# Autodesk Inventor assembly: mesa_0001_00001
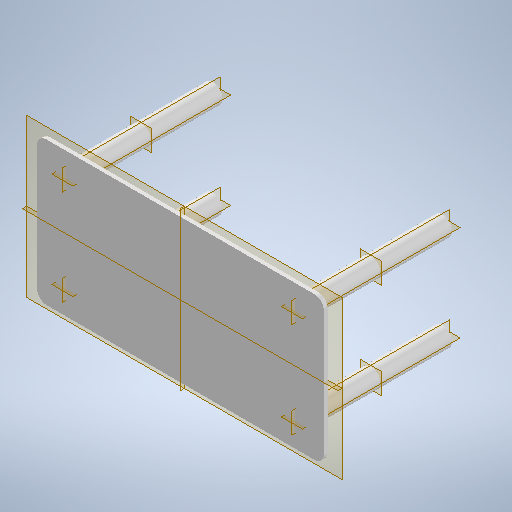
[picture p0: Inventor's stored thumbnail of the model, 512x512]
Saved by Autodesk Inventor 2025.2 (Build 292293000, 293)
## iProperties
Created: 2025-03-28
Part Number: mesa_0001_00001
Document SubType Name: Assembly
Designer: kenne
Author: kenne
## Documents named in this file (3)
- C:\Users\kenne\OneDrive\Ambiente de Trabalho\Robotica & Automação\Sistemas de Microcontroladores\Learning\Inventor\Exercices\Mesa\mesa_0001_00001.iam
- C:\Users\kenne\OneDrive\Ambiente de Trabalho\Robotica & Automação\Sistemas de Microcontroladores\Learning\Inventor\Exercices\Mesa\mesa_0001_00001.ipt
- C:\Users\kenne\OneDrive\Ambiente de Trabalho\Robotica & Automação\Sistemas de Microcontroladores\Learning\Inventor\Exercices\Mesa\pernas_0001_00001.ipt
## Components (5 placed, 2 different names)
1. mesa_0001_00001:1 — Flush:1, Flush:2, Flush:3, Mate:1, Flush:4, Flush:5
2. pernas_0001_00001:1 — Flush:7, Flush:9, Flush:10, Flush:11, Symmetry:1, Flush:14, Flush:15, Symmetry:2, Flush:16, Flush:17, Symmetry:3
3. pernas_0001_00001:2 — Flush:8, Flush:10, Flush:13, Flush:16, Symmetry:3
4. pernas_0001_00001:3 — Mate:1, Flush:4, Flush:5, Flush:6, Flush:7, Flush:8, Flush:12, Flush:13, Symmetry:1
5. pernas_0001_00001:4 — Flush:6, Flush:9, Flush:11, Flush:12, Flush:14, Flush:15, Symmetry:2, Flush:17
## Relationships (21: Flush 17, Symmetry 3, Mate 1)
- Flush:1: mesa_0001_00001:1
- Flush:2: mesa_0001_00001:1
- Flush:3: mesa_0001_00001:1
- Mate:1: mesa_0001_00001:1 ↔ pernas_0001_00001:3
- Flush:4 (600 mm): mesa_0001_00001:1 ↔ pernas_0001_00001:3
- Flush:5 (250 mm): mesa_0001_00001:1 ↔ pernas_0001_00001:3
- Flush:6: pernas_0001_00001:3 ↔ pernas_0001_00001:4
- Flush:7: pernas_0001_00001:1 ↔ pernas_0001_00001:3
- Flush:8: pernas_0001_00001:2 ↔ pernas_0001_00001:3
- Flush:9: pernas_0001_00001:1 ↔ pernas_0001_00001:4
- Flush:10: pernas_0001_00001:1 ↔ pernas_0001_00001:2
- Flush:11: pernas_0001_00001:1 ↔ pernas_0001_00001:4
- Flush:12: pernas_0001_00001:3 ↔ pernas_0001_00001:4
- Flush:13: pernas_0001_00001:2 ↔ pernas_0001_00001:3
- Symmetry:1: pernas_0001_00001:1 ↔ pernas_0001_00001:3
- Flush:14: pernas_0001_00001:1 ↔ pernas_0001_00001:4
- Flush:15: pernas_0001_00001:1 ↔ pernas_0001_00001:4
- Symmetry:2: pernas_0001_00001:1 ↔ pernas_0001_00001:4
- Flush:16: pernas_0001_00001:1 ↔ pernas_0001_00001:2
- Flush:17: pernas_0001_00001:1 ↔ pernas_0001_00001:4
- Symmetry:3: pernas_0001_00001:1 ↔ pernas_0001_00001:2
